# Autodesk Inventor assembly: Cylinder_Assembly_Final
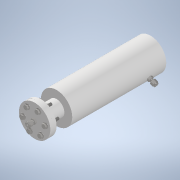
[picture p0: Inventor's stored thumbnail of the model, 180x180]
Saved by Autodesk Inventor 2022 (Build 260153000, 153)
## iProperties
Created: 2022-03-15
Part Number: Cylinder_Assembly_Final
Document SubType Name: Assembly
Designer: karee
Author: karee
## Documents named in this file (6)
- C:\Users\karee\OneDrive\Desktop\Cylinder_Assembly_Final.iam
- C:\Users\karee\OneDrive\Desktop\cylinder to be assembled.ipt
- C:\Users\karee\OneDrive\Desktop\flange2.ipt
- C:\Users\karee\OneDrive\Documents\Inventor\Content Center Files\R2022\en-US\JIS B 1189\JIS B 1189 - M8 x 1 - 40.ipt
- C:\Users\karee\OneDrive\Documents\Inventor\Content Center Files\R2022\en-US\ANSI B18.2.4.2M\ANSI B18.2.4.2M - M8x1.25 - 13.ipt
- C:\Users\karee\OneDrive\Documents\Inventor\Content Center Files\R2022\en-US\Parker A(26)\Parker A-Lok Male Taper Thread - Fractional Tube 1_4 x 1_4 (1).ipt
## Components (16 placed, 5 different names)
1. cylinder to be assembled:1 — Mate:1, Mate:2, Mate:4, Mate:6, Mate:8, Mate:10, Mate:12, Mate:14, Mate:15, Mate:18
2. flange2:1 — Mate:1, Mate:2, Insert:1, Insert:2, Insert:3, Insert:4, Insert:5, Insert:6, Mate:16, Mate:17
3. JIS B 1189 - Metric M8 x 1 x 40:1 — Insert:1, Mate:11
4. JIS B 1189 - Metric M8 x 1 x 40:2 — Insert:2, Mate:3
5. JIS B 1189 - Metric M8 x 1 x 40:3 — Insert:3, Mate:5
6. JIS B 1189 - Metric M8 x 1 x 40:4 — Insert:4, Mate:7
7. JIS B 1189 - Metric M8 x 1 x 40:5 — Insert:5, Mate:13, Mate:15
8. JIS B 1189 - Metric M8 x 1 x 40:6 — Insert:6, Mate:9
9. ANSI B18.2.4.2M M8x1.25:1 — Mate:3, Mate:4
10. ANSI B18.2.4.2M M8x1.25:2 — Mate:5, Mate:6
11. ANSI B18.2.4.2M M8x1.25:3 — Mate:7, Mate:8
12. ANSI B18.2.4.2M M8x1.25:4 — Mate:9, Mate:10
13. ANSI B18.2.4.2M M8x1.25:5 — Mate:11, Mate:12
14. ANSI B18.2.4.2M M8x1.25:6 — Mate:13, Mate:14
15. Parker A-Lok Male Taper Thread - Fractional Tube 1/4 x 1/4:1 — Mate:18
16. Parker A-Lok Male Taper Thread - Fractional Tube 1/4 x 1/4:2 — Mate:16, Mate:17
## Relationships (24: Mate 18, Insert 6)
- Mate:1: cylinder to be assembled:1 ↔ flange2:1
- Mate:2: cylinder to be assembled:1 ↔ flange2:1
- Insert:1: flange2:1 ↔ JIS B 1189 - Metric M8 x 1 x 40:1
- Insert:2: flange2:1 ↔ JIS B 1189 - Metric M8 x 1 x 40:2
- Insert:3: flange2:1 ↔ JIS B 1189 - Metric M8 x 1 x 40:3
- Insert:4: flange2:1 ↔ JIS B 1189 - Metric M8 x 1 x 40:4
- Insert:5: flange2:1 ↔ JIS B 1189 - Metric M8 x 1 x 40:5
- Insert:6: flange2:1 ↔ JIS B 1189 - Metric M8 x 1 x 40:6
- Mate:3: JIS B 1189 - Metric M8 x 1 x 40:2 ↔ ANSI B18.2.4.2M M8x1.25:1
- Mate:4: cylinder to be assembled:1 ↔ ANSI B18.2.4.2M M8x1.25:1
- Mate:5: JIS B 1189 - Metric M8 x 1 x 40:3 ↔ ANSI B18.2.4.2M M8x1.25:2
- Mate:6: cylinder to be assembled:1 ↔ ANSI B18.2.4.2M M8x1.25:2
- Mate:7: JIS B 1189 - Metric M8 x 1 x 40:4 ↔ ANSI B18.2.4.2M M8x1.25:3
- Mate:8: cylinder to be assembled:1 ↔ ANSI B18.2.4.2M M8x1.25:3
- Mate:9: JIS B 1189 - Metric M8 x 1 x 40:6 ↔ ANSI B18.2.4.2M M8x1.25:4
- Mate:10: cylinder to be assembled:1 ↔ ANSI B18.2.4.2M M8x1.25:4
- Mate:11: JIS B 1189 - Metric M8 x 1 x 40:1 ↔ ANSI B18.2.4.2M M8x1.25:5
- Mate:12: cylinder to be assembled:1 ↔ ANSI B18.2.4.2M M8x1.25:5
- Mate:13: JIS B 1189 - Metric M8 x 1 x 40:5 ↔ ANSI B18.2.4.2M M8x1.25:6
- Mate:14: cylinder to be assembled:1 ↔ ANSI B18.2.4.2M M8x1.25:6
- Mate:15: cylinder to be assembled:1 ↔ JIS B 1189 - Metric M8 x 1 x 40:5
- Mate:16: flange2:1 ↔ Parker A-Lok Male Taper Thread - Fractional Tube 1/4 x 1/4:2
- Mate:17: flange2:1 ↔ Parker A-Lok Male Taper Thread - Fractional Tube 1/4 x 1/4:2
- Mate:18: cylinder to be assembled:1 ↔ Parker A-Lok Male Taper Thread - Fractional Tube 1/4 x 1/4:1
